# Autodesk Inventor assembly: Assembly_HCMUTE-CDT23-CYLINDER
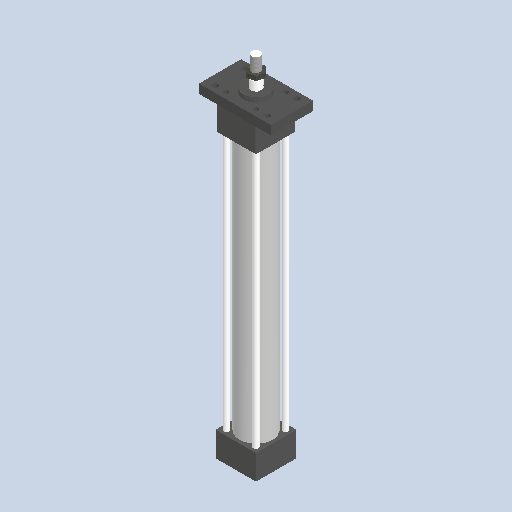
[picture p0: Inventor's stored thumbnail of the model, 512x512]
Saved by Autodesk Inventor 2023 (Build 270158000, 158)
## iProperties
Created: 2023-03-30
Part Number: Assembly_HCMUTE-CDT23-CYLINDER
Document SubType Name: Assembly
Designer: havie
Sending System: SolidWorks 2013
Last Author: win7
Last Saved: 2023-03-30
Author: havie
## Documents named in this file (9)
- D:\DO_AN_CDT\1.1. PART\Part_Cylinder\Assembly_HCMUTE-CDT23-CYLINDER-AIRTAC_SC32X300.iam
- D:\DO_AN_CDT\1.PART\Part_Cylinder\2309HCMUTE-CDT23-NAP_DUOI.ipt
- D:\DO_AN_CDT\1.PART\Part_Cylinder\2309HCMUTE-CDT23_COVER.ipt
- D:\DO_AN_CDT\1.PART\Part_Cylinder\2309HCMUTE-CDT23-NAP_DAU.ipt
- D:\DO_AN_CDT\1.PART\Part_Cylinder\2309HCMUTE-CDT23-PISTON.ipt
- D:\DO_AN_CDT\1.PART\Part_Cylinder\2309HCMUTE-CDT23-MAIN_SHAFT.ipt
- D:\DO_AN_CDT\1.PART\Part_Cylinder\2309HCMUTE-CDT23-TRUC_DINH_VI.ipt
- C:\Users\havie\Documents\Inventor\Content Center Files\R2023\en-US\ISO 4036(2)\ISO 4036 - M10(2).ipt
- D:\DO_AN_CDT\1.PART\Part_Cylinder\2309HCMUTE-CDT23-GA_SC32.ipt
## Components (11 placed, 8 different names)
1. 2309HCMUTE-CDT23_COVER:1 — Mate:1, Mate:3, Mate:5, Mate:6, Mate:8
2. 2309HCMUTE-CDT23-MAIN_SHAFT:1 — Mate:7, Mate:8, Mate:18, Flush:2, Flush:3, Flush:4
3. 2309HCMUTE-CDT23-NAP_DAU:1 — Mate:3, Angle:1, Mate:5, Mate:10, Mate:11, Mate:12, Mate:13, Mate:14, Mate:15, Mate:16, Flush:4, Mate:19, Mate:20, Mate:21
4. 2309HCMUTE-CDT23-NAP_DUOI:1 — Mate:1, Angle:1, Mate:6, Mate:9
5. 2309HCMUTE-CDT23-PISTON:1 — Mate:7, Flush:3
6. 2309HCMUTE-CDT23-TRUC_DINH_VI:1 — Mate:13, Mate:15
7. 2309HCMUTE-CDT23-TRUC_DINH_VI:2 — Mate:9, Mate:10
8. 2309HCMUTE-CDT23-TRUC_DINH_VI:3 — Mate:12, Mate:16
9. 2309HCMUTE-CDT23-TRUC_DINH_VI:4 — Mate:11, Mate:14
10. ISO 4036 M10:1 — Mate:18, Flush:2
11. 2309HCMUTE-CDT23-GA_SC32:1 — Mate:19, Mate:20, Mate:21
## Relationships (22: Mate 18, Flush 3, Angle 1)
- Mate:1: 2309HCMUTE-CDT23_COVER:1 ↔ 2309HCMUTE-CDT23-NAP_DUOI:1
- Mate:3: 2309HCMUTE-CDT23_COVER:1 ↔ 2309HCMUTE-CDT23-NAP_DAU:1
- Angle:1 (0 deg): 2309HCMUTE-CDT23-NAP_DAU:1 ↔ 2309HCMUTE-CDT23-NAP_DUOI:1
- Mate:5: 2309HCMUTE-CDT23_COVER:1 ↔ 2309HCMUTE-CDT23-NAP_DAU:1
- Mate:6: 2309HCMUTE-CDT23_COVER:1 ↔ 2309HCMUTE-CDT23-NAP_DUOI:1
- Mate:7: 2309HCMUTE-CDT23-MAIN_SHAFT:1 ↔ 2309HCMUTE-CDT23-PISTON:1
- Mate:8: 2309HCMUTE-CDT23_COVER:1 ↔ 2309HCMUTE-CDT23-MAIN_SHAFT:1
- Mate:9: 2309HCMUTE-CDT23-NAP_DUOI:1 ↔ 2309HCMUTE-CDT23-TRUC_DINH_VI:2
- Mate:10 (-10 mm): 2309HCMUTE-CDT23-NAP_DAU:1 ↔ 2309HCMUTE-CDT23-TRUC_DINH_VI:2
- Mate:11: 2309HCMUTE-CDT23-NAP_DAU:1 ↔ 2309HCMUTE-CDT23-TRUC_DINH_VI:4
- Mate:12: 2309HCMUTE-CDT23-NAP_DAU:1 ↔ 2309HCMUTE-CDT23-TRUC_DINH_VI:3
- Mate:13: 2309HCMUTE-CDT23-NAP_DAU:1 ↔ 2309HCMUTE-CDT23-TRUC_DINH_VI:1
- Mate:14 (-10 mm): 2309HCMUTE-CDT23-NAP_DAU:1 ↔ 2309HCMUTE-CDT23-TRUC_DINH_VI:4
- Mate:15 (-10 mm): 2309HCMUTE-CDT23-NAP_DAU:1 ↔ 2309HCMUTE-CDT23-TRUC_DINH_VI:1
- Mate:16 (-10 mm): 2309HCMUTE-CDT23-NAP_DAU:1 ↔ 2309HCMUTE-CDT23-TRUC_DINH_VI:3
- Mate:18: 2309HCMUTE-CDT23-MAIN_SHAFT:1 ↔ ISO 4036 M10:1
- Flush:2 (15 mm): 2309HCMUTE-CDT23-MAIN_SHAFT:1 ↔ ISO 4036 M10:1
- Flush:3: 2309HCMUTE-CDT23-MAIN_SHAFT:1 ↔ 2309HCMUTE-CDT23-PISTON:1
- Flush:4 (-32 mm): 2309HCMUTE-CDT23-MAIN_SHAFT:1 ↔ 2309HCMUTE-CDT23-NAP_DAU:1
- Mate:19: 2309HCMUTE-CDT23-NAP_DAU:1 ↔ 2309HCMUTE-CDT23-GA_SC32:1
- Mate:20: 2309HCMUTE-CDT23-NAP_DAU:1 ↔ 2309HCMUTE-CDT23-GA_SC32:1
- Mate:21: 2309HCMUTE-CDT23-NAP_DAU:1 ↔ 2309HCMUTE-CDT23-GA_SC32:1
